# Autodesk Inventor assembly: Shooter Assembly v2
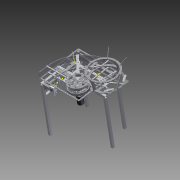
[picture p0: Inventor's stored thumbnail of the model, 180x180]
Saved by Autodesk Inventor 2013 (Build 170138000, 138)
## iProperties
Created: 2013-01-15
Part Number: Shooter Assembly v2
Document SubType Name: Assembly
Designer: actoennies
Mass: 8178.86 g
Surface Area: 23540.8 cm^2
Volume: 3991.15 cm^3
Density: 2.04925 g/cm^3
Author: actoennies
## Documents named in this file (37)
- C:\Users\Moses\Documents\GitHub\frc2013CAD\Launcher\Shooter\Shooter Assembly v2.iam
- C:\Users\Moses\Documents\GitHub\frc2013CAD\Launcher\Shooter\Bearing Mount v1.ipt
- C:\Users\Moses\Documents\GitHub\frc2013CAD\Launcher\Shooter\Outer Rail v1.ipt
- C:\Users\Moses\Documents\GitHub\frc2013CAD\Launcher\Shooter\Runner Rails v2.ipt
- C:\Users\Moses\Documents\GitHub\frc2013CAD\Launcher\Shooter\Bearing.ipt
- C:\Users\Moses\Documents\GitHub\frc2013CAD\Launcher\Shooter\Flywheel Assembly.iam
- C:\Users\Moses\Documents\GitHub\frc2013CAD\Launcher\Shooter\Shooter Mounter.ipt
- C:\Users\Moses\Documents\GitHub\frc2013CAD\Launcher\Shooter\Bearing Mount 2 v1.ipt
- C:\Users\Moses\Documents\GitHub\frc2013CAD\Launcher\Shooter\Shorter Shaft.ipt
- C:\Users\Moses\Documents\GitHub\frc2013CAD\Launcher\Shooter\Spacer Rube.ipt
- C:\Users\Moses\Documents\GitHub\frc2013CAD\Launcher\Shooter\Edge Mount.ipt
- C:\Users\Moses\Documents\GitHub\frc2013CAD\Launcher\Shooter\Square Tube.ipt
- C:\Users\Moses\Documents\GitHub\frc2013CAD\Launcher\Shooter\Flange Bearing Mount Tower.ipt
- C:\Users\Moses\Documents\GitHub\frc2013CAD\Launcher\Shooter\Flange Bearing Mount Tower Mirror.ipt
- C:\Users\Moses\Documents\GitHub\frc2013CAD\Launcher\Shooter\Bearing Mount Top.ipt
- C:\Users\Moses\Documents\GitHub\frc2013CAD\Launcher\Shooter\Square Motor Mount.ipt
- C:\Users\Moses\Documents\GitHub\frc2013CAD\Launcher\Hopper\HopperAssembly42inch_v5.iam
- C:\Users\Moses\Documents\GitHub\frc2013CAD\Launcher\Shooter\Shooter Assembly v2\Design Accelerator\Spur Gears1.iam
- C:\Users\Moses\Documents\GitHub\frc2013CAD\Launcher\Parts\Imported Components\Snow Blower Motor\Snow Blower Motor.iam
- C:\Users\Moses\Documents\GitHub\frc2013CAD\Launcher\Shooter\Snowblower Motor Mount.ipt
- C:\Users\Moses\Documents\GitHub\frc2013CAD\Launcher\Shooter\8mm shaft.ipt
- C:\Users\Moses\Documents\GitHub\frc2013CAD\Launcher\Shooter\CIM Bearing.ipt
- C:\Users\Moses\Documents\GitHub\frc2013CAD\Launcher\Parts\8 Plaction Wheel.iam
- C:\Users\Moses\Documents\GitHub\frc2013CAD\Launcher\Shooter\Square Tube 2.ipt
- C:\Users\Moses\Documents\GitHub\frc2013CAD\Launcher\Parts\CIM Motor\Motors_FR801-001.iam
- C:\Users\Moses\Documents\GitHub\frc2013CAD\Launcher\Shooter\Cim Mount.ipt
- C:\Users\Moses\Documents\GitHub\frc2013CAD\Launcher\Shooter\Hub v1.ipt
- C:\Users\Moses\Documents\GitHub\frc2013CAD\Launcher\Shooter\Camera Traffic Light Mount.ipt
- C:\Users\Moses\Documents\GitHub\frc2013CAD\Launcher\Shooter\Camera Gusset Plat.ipt
- C:\Users\Moses\Documents\GitHub\frc2013CAD\Launcher\Shooter\Square Tube 3.ipt
- C:\Users\Moses\Documents\GitHub\frc2013CAD\Launcher\Shooter\edge mount shortened.ipt
- C:\Users\Moses\Documents\GitHub\frc2013CAD\Launcher\Shooter\Camera.ipt
- C:\Users\Moses\Documents\GitHub\frc2013CAD\Launcher\Shooter\Square Tube 6.ipt
- C:\Users\Moses\Documents\GitHub\frc2013CAD\Launcher\Parts\NR-025_5-D(F,D-770).iam
- C:\Users\Moses\Documents\GitHub\frc2013CAD\Launcher\Shooter\Cylinder Mount.ipt
- C:\Users\Moses\Documents\GitHub\frc2013CAD\Launcher\Shooter\Cylinder Mount 2.ipt
- C:\Users\Moses\Documents\GitHub\frc2013CAD\Launcher\Shooter\Gusset Connector.ipt
## Components (46 placed, 36 different names)
1. Bearing Mount v1:1 — Insert:12, Insert:13, Insert:14, Insert:15, Insert:26, Insert:27, Mate:62, Mate:63
2. Outer Rail v1:1 — Insert:12, Insert:13, Insert:47, Insert:48, Flush:21, Mate:87
3. Runner Rails v2:1 — Insert:14, Insert:15, Mate:42
4. Flywheel Assembly:1 [sub-assembly] — Mate:61, Flush:30, Mate:68, Flush:31
5. Shooter Mounter:1 — Insert:26, Insert:27, Insert:34, Flush:11, Insert:35, Insert:36, Insert:37, Insert:38, Flush:19, Mate:45, Flush:24, Flush:40, Angle:6
6. Spacer Rube:1 — Insert:34, Flush:11
7. Bearing Mount 2 v1:1 — Insert:37, Insert:38, Insert:40
8. Bearing Mount 2 v1:2 — Insert:35, Insert:36, Insert:39
9. Bearing:3 — Insert:40, Flush:13, Mate:14, Mate:15
10. Bearing:4 — Insert:39, Flush:12, Mate:12, Mate:13, Mate:36, Mate:44
11. Shorter Shaft:1 — Flush:12, Mate:12, Mate:13, Mate:37
12. Shorter Shaft:2 — Flush:13, Mate:14, Mate:15, Mate:38
13. Edge Mount:2 — Flush:34, Mate:104, Flush:48, Mate:105, Mate:106, Flush:51, Flush:52
14. Square Tube:2 — Insert:41, Insert:42, Flush:19, Flush:23, Mate:52, Flush:27, Mate:81, Flush:32, Mate:93, Flush:41, Flush:42, Mate:125, Mate:126, Mate:130, Flush:50
15. Flange Bearing Mount Tower:1 — Insert:41, Insert:42, Insert:43
16. Bearing:5 — Insert:43, Mate:36, Mate:37
17. Flange Bearing Mount Tower Mirror:1 — Flush:55, Flush:56, Mate:135, Insert:59
18. Bearing:6 — Mate:38, Insert:59
19. Bearing Mount Top:1 — Insert:47, Insert:48, Mate:65, Mate:66, Mate:68
20. Square Motor Mount:1 — Flush:23, Mate:47, Mate:51, Flush:27, Mate:131
21. HopperAssembly42inch_v5:1 [sub-assembly] — Mate:42, Flush:21, Mate:87, Insert:60, Angle:4
22. Spur Gears:1 [sub-assembly] — Mate:44, Mate:45, Flush:24, Flush:25, Mate:46, Angle:2
23. Snow Blower Motor:1 [sub-assembly] — Flush:25, Mate:46, Angle:2, Insert:50, Insert:51
24. Snowblower Motor Mount:1 — Insert:50, Insert:51, Mate:47, Mate:51, Mate:52
25. 8mm shaft:1 — Mate:61, Flush:30, Mate:67, Flush:31, Mate:82, Mate:83, Mate:84, Mate:86
26. CIM Bearing:1 — Mate:65, Mate:66, Mate:67
27. CIM Bearing:2 — Mate:62, Mate:63, Insert:56
28. 8 Plaction Wheel:1 [sub-assembly] — Mate:88, Mate:89, Mate:90, Mate:91, Mate:92
29. Square Tube 2:1 — Mate:81, Flush:32, Flush:34, Mate:106, Mate:107, Mate:124, Flush:49, Mate:126, Flush:56
30. Motors_FR801-001:1 [sub-assembly] — Mate:82, Mate:83, Mate:84, Mate:143, Mate:144, Mate:145
31. Cim Mount:1 — Flush:40, Mate:143, Mate:144, Mate:145
32. Hub v1:1 — Mate:88, Mate:89, Mate:90, Flush:38
33. Hub v1:2 — Mate:91, Flush:38, Mate:92, Insert:56
34. Camera Traffic Light Mount:1 — Mate:93, Flush:41, Flush:42, Mate:94, Flush:43, Mate:127, Mate:128, Mate:129
35. Camera Gusset Plat:1 — Mate:94, Flush:43, Mate:133
36. Square Tube 3:1 — Mate:104, Flush:48, Mate:105, Mate:107, Mate:132, Flush:55, Mate:135, Mate:146, Flush:58, Flush:59, Angle:6
37. edge mount shortened:1 — Mate:124, Mate:125, Flush:49
38. Camera:1 — Mate:127, Mate:128, Mate:129
39. Edge Mount:3 — Mate:130, Mate:131, Flush:50, Mate:133
40. Edge Mount:4 — Mate:132, Flush:51, Flush:52, Mate:134, Flush:53, Flush:54
41. Square Tube 6:1 — Mate:134, Flush:53, Flush:54, Flush:57, Mate:147, Flush:60
42. NR-025_5-D(F,D-770):1 [sub-assembly] — Insert:60, Angle:4, Mate:136, Mate:137, Mate:138, Mate:139, Mate:140
43. Cylinder Mount:1 — Mate:136, Mate:137, Mate:138, Angle:5
44. Cylinder Mount 2:1 — Mate:139, Mate:140, Angle:5
45. Gusset Connector:1 — Mate:147, Flush:59, Flush:60
46. Gusset Connector:2 — Mate:146, Flush:57, Flush:58
## Relationships (118: Mate 60, Flush 31, Insert 23, Angle 4)
- Insert:12: Bearing Mount v1:1 ↔ Outer Rail v1:1
- Insert:13: Bearing Mount v1:1 ↔ Outer Rail v1:1
- Insert:14: Bearing Mount v1:1 ↔ Runner Rails v2:1
- Insert:15: Bearing Mount v1:1 ↔ Runner Rails v2:1
- Insert:26: Bearing Mount v1:1 ↔ Shooter Mounter:1
- Insert:27: Bearing Mount v1:1 ↔ Shooter Mounter:1
- Insert:34: Shooter Mounter:1 ↔ Spacer Rube:1
- Flush:11: Shooter Mounter:1 ↔ Spacer Rube:1
- Insert:35: Shooter Mounter:1 ↔ Bearing Mount 2 v1:2
- Insert:36: Shooter Mounter:1 ↔ Bearing Mount 2 v1:2
- Insert:37: Shooter Mounter:1 ↔ Bearing Mount 2 v1:1
- Insert:38: Shooter Mounter:1 ↔ Bearing Mount 2 v1:1
- Insert:39: Bearing Mount 2 v1:2 ↔ Bearing:4
- Insert:40: Bearing Mount 2 v1:1 ↔ Bearing:3
- Flush:12 (-25.4 mm): Bearing:4 ↔ Shorter Shaft:1
- Mate:12: Bearing:4 ↔ Shorter Shaft:1
- Mate:13: Bearing:4 ↔ Shorter Shaft:1
- Flush:13 (-25.4 mm): Bearing:3 ↔ Shorter Shaft:2
- Mate:14: Bearing:3 ↔ Shorter Shaft:2
- Mate:15: Bearing:3 ↔ Shorter Shaft:2
- Insert:41: Square Tube:2 ↔ Flange Bearing Mount Tower:1
- Insert:42: Square Tube:2 ↔ Flange Bearing Mount Tower:1
- Insert:43: Flange Bearing Mount Tower:1 ↔ Bearing:5
- Flush:19: Shooter Mounter:1 ↔ Square Tube:2
- Mate:36: Bearing:4 ↔ Bearing:5
- Mate:37: Shorter Shaft:1 ↔ Bearing:5
- Mate:38: Shorter Shaft:2 ↔ Bearing:6
- Insert:47: Outer Rail v1:1 ↔ Bearing Mount Top:1
- Insert:48: Outer Rail v1:1 ↔ Bearing Mount Top:1
- Mate:42: Runner Rails v2:1 ↔ HopperAssembly42inch_v5:1
- Flush:21: Outer Rail v1:1 ↔ HopperAssembly42inch_v5:1
- Flush:23 (152.4 mm): Square Tube:2 ↔ Square Motor Mount:1
- Mate:44: Bearing:4 ↔ Spur Gears:1
- Mate:45 (25.4 mm): Shooter Mounter:1 ↔ Spur Gears:1
- Flush:24: Shooter Mounter:1 ↔ Spur Gears:1
- Flush:25 (-3.175 mm): Spur Gears:1 ↔ Snow Blower Motor:1
- Mate:46: Spur Gears:1 ↔ Snow Blower Motor:1
- Angle:2 (0 deg): Spur Gears:1 ↔ Snow Blower Motor:1
- Insert:50: Snow Blower Motor:1 ↔ Snowblower Motor Mount:1
- Insert:51: Snow Blower Motor:1 ↔ Snowblower Motor Mount:1
- Mate:47: Square Motor Mount:1 ↔ Snowblower Motor Mount:1
- Mate:51: Square Motor Mount:1 ↔ Snowblower Motor Mount:1
- Mate:52: Square Tube:2 ↔ Snowblower Motor Mount:1
- Flush:27: Square Tube:2 ↔ Square Motor Mount:1
- Mate:61: Flywheel Assembly:1 ↔ 8mm shaft:1
- Flush:30 (12.7 mm): Flywheel Assembly:1 ↔ 8mm shaft:1
- Mate:62: Bearing Mount v1:1 ↔ CIM Bearing:2
- Mate:63: Bearing Mount v1:1 ↔ CIM Bearing:2
- Mate:65: Bearing Mount Top:1 ↔ CIM Bearing:1
- Mate:66: Bearing Mount Top:1 ↔ CIM Bearing:1
- Mate:67: 8mm shaft:1 ↔ CIM Bearing:1
- Mate:68 (6.35 mm): Flywheel Assembly:1 ↔ Bearing Mount Top:1
- Flush:31: Flywheel Assembly:1 ↔ 8mm shaft:1
- Mate:81: Square Tube:2 ↔ Square Tube 2:1
- Flush:32: Square Tube:2 ↔ Square Tube 2:1
- Flush:34: Edge Mount:2 ↔ Square Tube 2:1
- Mate:82: 8mm shaft:1 ↔ Motors_FR801-001:1
- Mate:83: 8mm shaft:1 ↔ Motors_FR801-001:1
- Mate:84: 8mm shaft:1 ↔ Motors_FR801-001:1
- Mate:86: 8mm shaft:1
- Mate:87 (25.4 mm): Outer Rail v1:1 ↔ HopperAssembly42inch_v5:1
- Mate:88: 8 Plaction Wheel:1 ↔ Hub v1:1
- Mate:89: 8 Plaction Wheel:1 ↔ Hub v1:1
- Mate:90: 8 Plaction Wheel:1 ↔ Hub v1:1
- Mate:91: 8 Plaction Wheel:1 ↔ Hub v1:2
- Flush:38: Hub v1:1 ↔ Hub v1:2
- Mate:92: 8 Plaction Wheel:1 ↔ Hub v1:2
- Insert:56 (3.175 mm): CIM Bearing:2 ↔ Hub v1:2
- Flush:40: Shooter Mounter:1 ↔ Cim Mount:1
- Mate:93: Square Tube:2 ↔ Camera Traffic Light Mount:1
- Flush:41: Square Tube:2 ↔ Camera Traffic Light Mount:1
- Flush:42: Square Tube:2 ↔ Camera Traffic Light Mount:1
- Mate:94: Camera Traffic Light Mount:1 ↔ Camera Gusset Plat:1
- Flush:43 (11.1125 mm): Camera Traffic Light Mount:1 ↔ Camera Gusset Plat:1
- Mate:104: Edge Mount:2 ↔ Square Tube 3:1
- Flush:48: Edge Mount:2 ↔ Square Tube 3:1
- Mate:105: Edge Mount:2 ↔ Square Tube 3:1
- Mate:106: Edge Mount:2 ↔ Square Tube 2:1
- Mate:107: Square Tube 2:1 ↔ Square Tube 3:1
- Mate:124: Square Tube 2:1 ↔ edge mount shortened:1
- Mate:125: Square Tube:2 ↔ edge mount shortened:1
- Flush:49: Square Tube 2:1 ↔ edge mount shortened:1
- Mate:126: Square Tube:2 ↔ Square Tube 2:1
- Mate:127: Camera Traffic Light Mount:1 ↔ Camera:1
- Mate:128: Camera Traffic Light Mount:1 ↔ Camera:1
- Mate:129: Camera Traffic Light Mount:1 ↔ Camera:1
- Mate:130: Square Tube:2 ↔ Edge Mount:3
- Mate:131: Square Motor Mount:1 ↔ Edge Mount:3
- Flush:50: Square Tube:2 ↔ Edge Mount:3
- Mate:132: Square Tube 3:1 ↔ Edge Mount:4
- Flush:51 (247.65 mm): Edge Mount:2 ↔ Edge Mount:4
- Flush:52 (-95.25 mm): Edge Mount:2 ↔ Edge Mount:4
- Mate:133: Camera Gusset Plat:1 ↔ Edge Mount:3
- Mate:134: Edge Mount:4 ↔ Square Tube 6:1
- Flush:53: Edge Mount:4 ↔ Square Tube 6:1
- Flush:54: Edge Mount:4 ↔ Square Tube 6:1
- Flush:55: Flange Bearing Mount Tower Mirror:1 ↔ Square Tube 3:1
- Flush:56: Flange Bearing Mount Tower Mirror:1 ↔ Square Tube 2:1
- Mate:135: Flange Bearing Mount Tower Mirror:1 ↔ Square Tube 3:1
- Insert:59: Flange Bearing Mount Tower Mirror:1 ↔ Bearing:6
- Insert:60 (-6.35 mm): HopperAssembly42inch_v5:1 ↔ NR-025_5-D(F,D-770):1
- Angle:4 (180 deg): HopperAssembly42inch_v5:1 ↔ NR-025_5-D(F,D-770):1
- Mate:136: NR-025_5-D(F,D-770):1 ↔ Cylinder Mount:1
- Mate:137: NR-025_5-D(F,D-770):1 ↔ Cylinder Mount:1
- Mate:138: NR-025_5-D(F,D-770):1 ↔ Cylinder Mount:1
- Mate:139: NR-025_5-D(F,D-770):1 ↔ Cylinder Mount 2:1
- Mate:140: NR-025_5-D(F,D-770):1 ↔ Cylinder Mount 2:1
- Angle:5 (180 deg): Cylinder Mount:1 ↔ Cylinder Mount 2:1
- Mate:143: Motors_FR801-001:1 ↔ Cim Mount:1
- Mate:144: Motors_FR801-001:1 ↔ Cim Mount:1
- Mate:145: Motors_FR801-001:1 ↔ Cim Mount:1
- Mate:146: Square Tube 3:1 ↔ Gusset Connector:2
- Flush:57: Square Tube 6:1 ↔ Gusset Connector:2
- Flush:58: Square Tube 3:1 ↔ Gusset Connector:2
- Mate:147: Square Tube 6:1 ↔ Gusset Connector:1
- Flush:59: Square Tube 3:1 ↔ Gusset Connector:1
- Flush:60: Square Tube 6:1 ↔ Gusset Connector:1
- Angle:6 (0 deg): Shooter Mounter:1 ↔ Square Tube 3:1
